# Autodesk Inventor assembly: Assembly1
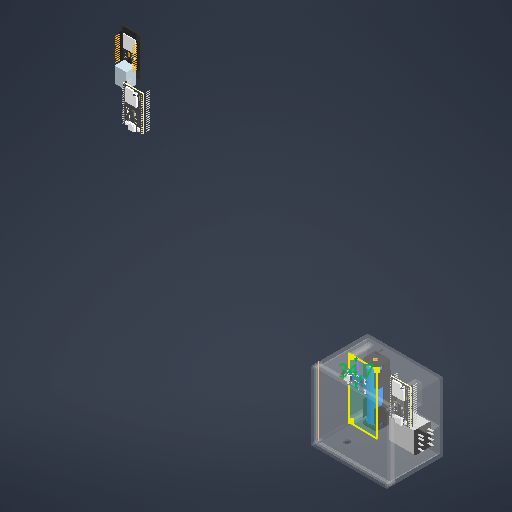
[picture p0: Inventor's stored thumbnail of the model, 512x512]
Saved by Autodesk Inventor 2027.1 (Build 311270010, 270A)
## iProperties
Created: 2026-09-21
Part Number: Assembly1
Document SubType Name: Assembly
Designer: LENOVO
Author: LENOVO
## Documents named in this file (9)
- C:\Users\LENOVO\OneDrive\Documents\PROJECK RISET\BOX_ALERT\Assembly1.iam
- C:\Users\LENOVO\Downloads\WT32-ESP01 v2\WT32-ESP01 v2.ipt
- C:\Users\LENOVO\Downloads\Battery Holder\Battery Holder.ipt
- C:\Users\LENOVO\Downloads\ESP32-DevkitC32U\ESP32-DevkitC32U.ipt
- C:\Users\LENOVO\OneDrive\Documents\PROJECK RISET\BOX_ALERT\alert.ipt
- C:\Users\LENOVO\Downloads\relay-my2n-2.snapshot.1\MY2\MY2.ipt
- C:\Users\LENOVO\OneDrive\Documents\PROJECK RISET\BOX_ALERT\box_alert.ipt
- C:\Users\LENOVO\OneDrive\Documents\PROJECK RISET\BOX_ALERT\tutup_box_alert.ipt
- C:\Users\LENOVO\Downloads\TP4056_Charging_Module_Type_C\TP4056_Charging_Module_Type_C.ipt
## Components (9 placed, 8 different names)
1. WT32-ESP01 v2:1
2. Battery Holder:1
3. ESP32-DevkitC32U:1
4. ESP32-DevkitC32U:2
5. alert:1
6. MY2:1
7. box_alert:1 — Flush:1, Flush:2
8. tutup_box_alert:1 — Flush:1, Flush:2
9. TP4056_Charging_Module_Type_C:1
## Relationships (2: Flush 2)
- Flush:1: box_alert:1 ↔ tutup_box_alert:1
- Flush:2: box_alert:1 ↔ tutup_box_alert:1
